# Autodesk Inventor assembly: X-AXIS ASSEMBLY
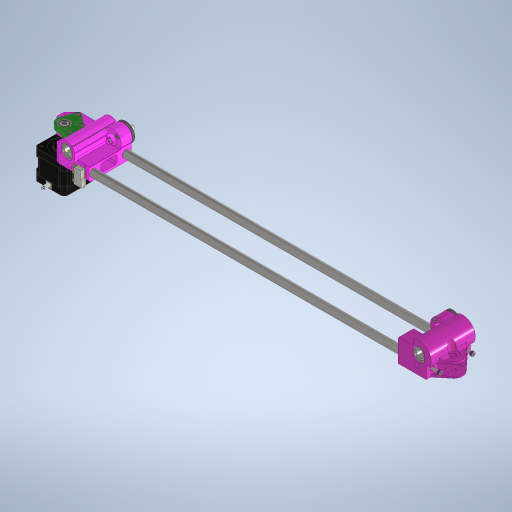
[picture p0: Inventor's stored thumbnail of the model, 512x512]
Saved by Autodesk Inventor 2023 (Build 270158000, 158)
## iProperties
Created: 2019-09-17
Part Number: X-AXIS ASSEMBLY
Document SubType Name: Assembly
Designer: pepd9
Author: pepd9
## Documents named in this file (21)
- D:\000 - PEPCORP CLOUD\00- Legacy\Designs\MK3PRO P1\X-Axis\X-AXIS ASSEMBLY.iam
- D:\000 - PEPCORP CLOUD\00- Legacy\Designs\MK3PRO P1\X-Axis\X-end-motor.ipt
- D:\000 - PEPCORP CLOUD\00- Legacy\Designs\MK3PRO P1\COMPONENTS\LM10UU.ipt
- D:\000 - PEPCORP CLOUD\00- Legacy\Designs\MK3PRO P1\X-Axis\x-end-idler(R2).ipt
- D:\000 - PEPCORP CLOUD\00- Legacy\Designs\MK3PRO P1\X-Axis\X-AXIS ROD.ipt
- D:\000 - PEPCORP CLOUD\00- Legacy\Designs\MK3PRO P1\COMPONENTS\M5 Nylock.ipt
- D:\000 - PEPCORP CLOUD\00- Legacy\Designs\MK3PRO P1\COMPONENTS\SHCS_M5_25.ipt
- D:\000 - PEPCORP CLOUD\00- Legacy\Designs\MK3PRO P1\COMPONENTS\Idler Roller, flat.ipt
- D:\000 - PEPCORP CLOUD\00- Legacy\Designs\MK3PRO P1\X-Axis\Z_NUT_1.ipt
- D:\000 - PEPCORP CLOUD\00- Legacy\Designs\MK3PRO P1\COMPONENTS\M3 Nut.ipt
- D:\000 - PEPCORP CLOUD\00- Legacy\Designs\MK3PRO P1\COMPONENTS\SHCS_M3_18.ipt
- D:\000 - PEPCORP CLOUD\00- Legacy\Designs\MK3PRO P1\X-Axis\x-axis-stepper-motor.iam
- D:\000 - PEPCORP CLOUD\00- Legacy\Designs\MK3PRO P1\COMPONENTS\GT2_16T.ipt
- D:\000 - PEPCORP CLOUD\00- Legacy\Designs\MK3PRO P1\COMPONENTS\625 Bearing.ipt
- D:\000 - PEPCORP CLOUD\00- Legacy\Designs\MK3PRO P1\X-Axis\X-Axis Motor Support.ipt
- D:\000 - PEPCORP CLOUD\00- Legacy\Designs\MK3PRO P1\COMPONENTS\NUT_SQUARE_M3.ipt
- D:\000 - PEPCORP CLOUD\00- Legacy\Designs\MK3PRO P1\COMPONENTS\SHCS_M3_20.ipt
- D:\000 - PEPCORP CLOUD\00- Legacy\Designs\MK3PRO P1\COMPONENTS\Small Limit Switch.iam
- D:\000 - PEPCORP CLOUD\00- Legacy\Designs\MK3PRO P1\COMPONENTS\SHCS_M3_10.ipt
- D:\000 - PEPCORP CLOUD\00- Legacy\Designs\MK3PRO P1\X-Axis\X-End-Idler-V0.2.ipt
- D:\000 - PEPCORP CLOUD\00- Legacy\Designs\MK3PRO P1\X-Axis\X-end-motor v0.2.ipt
## Components (41 placed, 20 different names)
1. X-end-motor:1 — Mate:1, Mate:2, Mate:3, Flush:1, Mate:7, Mate:8, Mate:9, Mate:10, Mate:13, Mate:21, Mate:22, Mate:23, Mate:31, Mate:32, Mate:33, Mate:34, Mate:39, Mate:43, Mate:44, Mate:45, Mate:49, Mate:58, Mate:59, Mate:85, Mate:86, Mate:87, Mate:88, Mate:89, Mate:90, Mate:91, Mate:92, Mate:93, Mate:102, Mate:103, Mate:104, Mate:105, Mate:108, Flush:6, Flush:7, Mate:109, Mate:110, Mate:111
2. LM10UU:1 — Mate:1, Mate:3
3. LM10UU:2 — Mate:6, Flush:2, Mate:113
4. LM10UU:3 — Mate:4, Mate:5
5. LM10UU:4 — Mate:2, Flush:1, Mate:115
6. x-end-idler(R2):1 — Mate:4, Mate:5, Mate:6, Flush:2, Mate:11, Mate:12, Mate:13, Mate:14, Mate:15, Mate:16, Mate:17, Mate:18, Mate:20, Mate:24, Mate:25, Mate:26, Mate:27, Mate:28, Mate:29, Mate:30, Mate:70, Mate:71, Mate:72, Mate:75, Flush:4, Mate:76, Mate:77, Flush:5, Angle:1, Mate:107
7. X-AXIS ROD:1 — Mate:8, Mate:9, Mate:12
8. X-AXIS ROD:2 — Mate:7, Mate:10, Mate:11, Mate:114, Mate:116
9. M5 Nylock:1 — Mate:15, Mate:16, Mate:17
10. SHCS_M5_25:1 — Mate:14, Mate:18, Mate:19
11. Idler Roller, flat:1 — Mate:19, Mate:20
12. Z_NUT_1:1 — Mate:21, Mate:22, Mate:23, Mate:40, Mate:41, Mate:42
13. Z_NUT_1:2 — Mate:24, Mate:25, Mate:26, Mate:35, Mate:36, Mate:37, Mate:38
14. M3 Nut:1 — Mate:31, Mate:32
15. M3 Nut:2 — Mate:33, Mate:34
16. M3 Nut:3 — Mate:27, Mate:28
17. M3 Nut:4 — Mate:29, Mate:30
18. SHCS_M3_18:1 — Mate:39, Mate:42
19. SHCS_M3_18:2 — Mate:40, Mate:41
20. SHCS_M3_18:3 — Mate:35, Mate:38
21. SHCS_M3_18:4 — Mate:36, Mate:37
22. x-axis-stepper-motor:1 [sub-assembly] — Mate:43, Mate:44, Mate:50, Mate:51, Mate:106
23. SHCS_M3_18:5 — Mate:45, Mate:49
24. GT2_16T:1 — Mate:50, Mate:51, Mate:112
25. M3 Nut:5 — Mate:58, Mate:59
26. NUT_SQUARE_M3:1 — Mate:70, Mate:71, Mate:72
27. NUT_SQUARE_M3:2 — Mate:75, Angle:1, Mate:107
28. SHCS_M3_20:1 — Mate:77, Flush:5
29. SHCS_M3_20:2 — Flush:4, Mate:76
30. X-Axis Motor Support:1 — Mate:85, Mate:86, Mate:87, Mate:95, Mate:96, Mate:97, Mate:98, Mate:99, Mate:100, Mate:101
31. M3 Nut:6 — Mate:88, Mate:89, Mate:90
32. M3 Nut:7 — Mate:91, Mate:92, Mate:93
33. 625 Bearing:1 — Mate:95, Mate:112
34. SHCS_M3_10:1 — Mate:96, Mate:98
35. SHCS_M3_10:2 — Mate:97, Mate:99
36. SHCS_M3_10:3 — Mate:100, Mate:101
37. SHCS_M3_18:6 — Mate:102, Mate:105, Mate:106
38. SHCS_M3_18:7 — Mate:103, Mate:104
39. Small Limit Switch:1 [sub-assembly] — Mate:109, Mate:110, Mate:111
40. X-End-Idler-V0.2:1 — Mate:113, Mate:114
41. X-end-motor v0.2:1 — Mate:115, Mate:116
## Relationships (94: Mate 87, Flush 6, Angle 1)
- Mate:1: X-end-motor:1 ↔ LM10UU:1
- Mate:2: X-end-motor:1 ↔ LM10UU:4
- Mate:3: X-end-motor:1 ↔ LM10UU:1
- Flush:1: X-end-motor:1 ↔ LM10UU:4
- Mate:4: LM10UU:3 ↔ x-end-idler(R2):1
- Mate:5: LM10UU:3 ↔ x-end-idler(R2):1
- Mate:6: LM10UU:2 ↔ x-end-idler(R2):1
- Flush:2: LM10UU:2 ↔ x-end-idler(R2):1
- Mate:7: X-end-motor:1 ↔ X-AXIS ROD:2
- Mate:8: X-end-motor:1 ↔ X-AXIS ROD:1
- Mate:9: X-end-motor:1 ↔ X-AXIS ROD:1
- Mate:10: X-end-motor:1 ↔ X-AXIS ROD:2
- Mate:11: x-end-idler(R2):1 ↔ X-AXIS ROD:2
- Mate:12: x-end-idler(R2):1 ↔ X-AXIS ROD:1
- Mate:13 (427 mm): X-end-motor:1 ↔ x-end-idler(R2):1
- Mate:14: x-end-idler(R2):1 ↔ SHCS_M5_25:1
- Mate:15: x-end-idler(R2):1 ↔ M5 Nylock:1
- Mate:16: x-end-idler(R2):1 ↔ M5 Nylock:1
- Mate:17: x-end-idler(R2):1 ↔ M5 Nylock:1
- Mate:18: x-end-idler(R2):1 ↔ SHCS_M5_25:1
- Mate:19: SHCS_M5_25:1 ↔ Idler Roller, flat:1
- Mate:20 (0.5 mm): x-end-idler(R2):1 ↔ Idler Roller, flat:1
- Mate:21: X-end-motor:1 ↔ Z_NUT_1:1
- Mate:22: X-end-motor:1 ↔ Z_NUT_1:1
- Mate:23: X-end-motor:1 ↔ Z_NUT_1:1
- Mate:24: x-end-idler(R2):1 ↔ Z_NUT_1:2
- Mate:25: x-end-idler(R2):1 ↔ Z_NUT_1:2
- Mate:26: x-end-idler(R2):1 ↔ Z_NUT_1:2
- Mate:27: x-end-idler(R2):1 ↔ M3 Nut:3
- Mate:28: x-end-idler(R2):1 ↔ M3 Nut:3
- Mate:29: x-end-idler(R2):1 ↔ M3 Nut:4
- Mate:30: x-end-idler(R2):1 ↔ M3 Nut:4
- Mate:31: X-end-motor:1 ↔ M3 Nut:1
- Mate:32: X-end-motor:1 ↔ M3 Nut:1
- Mate:33: X-end-motor:1 ↔ M3 Nut:2
- Mate:34: X-end-motor:1 ↔ M3 Nut:2
- Mate:35: Z_NUT_1:2 ↔ SHCS_M3_18:3
- Mate:36: Z_NUT_1:2 ↔ SHCS_M3_18:4
- Mate:37: Z_NUT_1:2 ↔ SHCS_M3_18:4
- Mate:38: Z_NUT_1:2 ↔ SHCS_M3_18:3
- Mate:39: X-end-motor:1 ↔ SHCS_M3_18:1
- Mate:40: Z_NUT_1:1 ↔ SHCS_M3_18:2
- Mate:41: Z_NUT_1:1 ↔ SHCS_M3_18:2
- Mate:42: Z_NUT_1:1 ↔ SHCS_M3_18:1
- Mate:43: X-end-motor:1 ↔ x-axis-stepper-motor:1
- Mate:44: X-end-motor:1 ↔ x-axis-stepper-motor:1
- Mate:45: X-end-motor:1 ↔ SHCS_M3_18:5
- Mate:49: X-end-motor:1 ↔ SHCS_M3_18:5
- Mate:50: x-axis-stepper-motor:1 ↔ GT2_16T:1
- Mate:51 (0.5 mm): x-axis-stepper-motor:1 ↔ GT2_16T:1
- Mate:58: X-end-motor:1 ↔ M3 Nut:5
- Mate:59: X-end-motor:1 ↔ M3 Nut:5
- Mate:70: x-end-idler(R2):1 ↔ NUT_SQUARE_M3:1
- Mate:71: x-end-idler(R2):1 ↔ NUT_SQUARE_M3:1
- Mate:72: x-end-idler(R2):1 ↔ NUT_SQUARE_M3:1
- Mate:75: x-end-idler(R2):1 ↔ NUT_SQUARE_M3:2
- Flush:4: x-end-idler(R2):1 ↔ SHCS_M3_20:2
- Mate:76: x-end-idler(R2):1 ↔ SHCS_M3_20:2
- Mate:77: x-end-idler(R2):1 ↔ SHCS_M3_20:1
- Flush:5: x-end-idler(R2):1 ↔ SHCS_M3_20:1
- Mate:85: X-end-motor:1 ↔ X-Axis Motor Support:1
- Mate:86: X-end-motor:1 ↔ X-Axis Motor Support:1
- Mate:87: X-end-motor:1 ↔ X-Axis Motor Support:1
- Mate:88: X-end-motor:1 ↔ M3 Nut:6
- Mate:89: X-end-motor:1 ↔ M3 Nut:6
- Mate:90: X-end-motor:1 ↔ M3 Nut:6
- Mate:91: X-end-motor:1 ↔ M3 Nut:7
- Mate:92: X-end-motor:1 ↔ M3 Nut:7
- Mate:93: X-end-motor:1 ↔ M3 Nut:7
- Mate:95: X-Axis Motor Support:1 ↔ 625 Bearing:1
- Mate:96: X-Axis Motor Support:1 ↔ SHCS_M3_10:1
- Mate:97: X-Axis Motor Support:1 ↔ SHCS_M3_10:2
- Mate:98: X-Axis Motor Support:1 ↔ SHCS_M3_10:1
- Mate:99: X-Axis Motor Support:1 ↔ SHCS_M3_10:2
- Mate:100: X-Axis Motor Support:1 ↔ SHCS_M3_10:3
- Mate:101: X-Axis Motor Support:1 ↔ SHCS_M3_10:3
- Mate:102: X-end-motor:1 ↔ SHCS_M3_18:6
- Mate:103: X-end-motor:1 ↔ SHCS_M3_18:7
- Mate:104: X-end-motor:1 ↔ SHCS_M3_18:7
- Mate:105: X-end-motor:1 ↔ SHCS_M3_18:6
- Mate:106: x-axis-stepper-motor:1 ↔ SHCS_M3_18:6
- Angle:1 (0 deg): x-end-idler(R2):1 ↔ NUT_SQUARE_M3:2
- Mate:107: x-end-idler(R2):1 ↔ NUT_SQUARE_M3:2
- Mate:108: X-end-motor:1
- Flush:6: X-end-motor:1
- Flush:7 (213.5 mm): X-end-motor:1
- Mate:109: X-end-motor:1 ↔ Small Limit Switch:1
- Mate:110: X-end-motor:1 ↔ Small Limit Switch:1
- Mate:111: X-end-motor:1 ↔ Small Limit Switch:1
- Mate:112 (0.5 mm): GT2_16T:1 ↔ 625 Bearing:1
- Mate:113: LM10UU:2 ↔ X-End-Idler-V0.2:1
- Mate:114: X-AXIS ROD:2 ↔ X-End-Idler-V0.2:1
- Mate:115: LM10UU:4 ↔ X-end-motor v0.2:1
- Mate:116: X-AXIS ROD:2 ↔ X-end-motor v0.2:1
